# Autodesk Inventor assembly: mascon-new
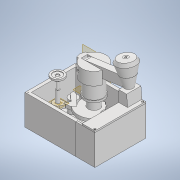
[picture p0: Inventor's stored thumbnail of the model, 180x180]
Saved by Autodesk Inventor 2021 (Build 250183000, 183)
## iProperties
Created: 2021-04-28
Part Number: mascon-new
Document SubType Name: Assembly
Designer: ben
Author: ben
## Documents named in this file (13)
- C:\Users\ars-admin\Documents\GitHub\r68-bve-mascon\mascon-new.iam
- C:\Users\ars-admin\Documents\GitHub\r68-bve-mascon\handle\handle.iam
- C:\Users\ars-admin\Documents\GitHub\r68-bve-mascon\shell\shell.iam
- C:\Users\ars-admin\Documents\GitHub\r68-bve-mascon\handle_base_rod.ipt
- C:\Users\ars-admin\Documents\GitHub\r68-bve-mascon\handle_base_potholder.ipt
- C:\Users\ars-admin\Documents\GitHub\r68-bve-mascon\handle_holder.ipt
- C:\Users\ars-admin\Documents\GitHub\r68-bve-mascon\Reverser.ipt
- C:\Users\ars-admin\Documents\GitHub\r68-bve-mascon\reverser-base.ipt
- C:\Users\ars-admin\Documents\GitHub\r68-bve-mascon\NotchClickerAsm.iam
- C:\Users\ars-admin\Documents\GitHub\r68-bve-mascon\ReverserNotch\ReverserClickAsm.iam
- C:\Users\ars-admin\Documents\GitHub\r68-bve-mascon\handle-base\handle_base.iam
- C:\Users\ars-admin\Documents\GitHub\r68-bve-mascon\handle_base2.ipt
- C:\Users\ars-admin\Documents\GitHub\r68-bve-mascon\misc\V-wheel.ipt
## Components (12 placed, 12 different names)
1. shell:1 [sub-assembly] — Flush:4, Mate:12, Mate:14, Mate:15, Rotational:2, Mate:22, Mate:23
2. handle_base_rod:1
3. handle_base_potholder:1 — Flush:9
4. handle_holder:1 — Rotational:1, Mate:16
5. Reverser:1 — Flush:4, Flush:5
6. reverser-base:1 — Flush:5, Flush:6, Flush:7, Flush:10
7. NotchClickerAsm:1 [sub-assembly] — Mate:12, Mate:20, Mate:21, Mate:22
8. ReverserClickAsm:1 [sub-assembly] — Mate:23
9. handle:1 [sub-assembly] — Rotational:1, Mate:17
10. handle_base:1 [sub-assembly] — Mate:14, Mate:15, Mate:16, Mate:17, Rotational:2, Mate:18, Flush:8, Mate:19
11. handle_base2:1 — Mate:18, Flush:8, Mate:19, Flush:9
12. V-wheel:1 — Mate:20, Mate:21
## Relationships (20: Mate 11, Flush 7, RevoluteJoint 2)
- Flush:4: shell:1 ↔ Reverser:1
- Flush:5: Reverser:1 ↔ reverser-base:1
- Mate:12: shell:1 ↔ NotchClickerAsm:1
- Flush:6 (-36.375 mm): reverser-base:1
- Flush:7: reverser-base:1
- Mate:14: shell:1 ↔ handle_base:1
- Mate:15: shell:1 ↔ handle_base:1
- Rotational:1 [RevoluteJoint]: handle_holder:1 ↔ handle:1
- Mate:16: handle_holder:1 ↔ handle_base:1
- Mate:17: handle:1 ↔ handle_base:1
- Rotational:2 [RevoluteJoint] (-5 mm): shell:1 ↔ handle_base:1
- Mate:18: handle_base:1 ↔ handle_base2:1
- Flush:8: handle_base:1 ↔ handle_base2:1
- Mate:19: handle_base:1 ↔ handle_base2:1
- Flush:9: handle_base_potholder:1 ↔ handle_base2:1
- Mate:20: NotchClickerAsm:1 ↔ V-wheel:1
- Mate:21: NotchClickerAsm:1 ↔ V-wheel:1
- Mate:22: shell:1 ↔ NotchClickerAsm:1
- Mate:23: shell:1 ↔ ReverserClickAsm:1
- Flush:10: reverser-base:1
